# Autodesk Inventor assembly: ArcadeController
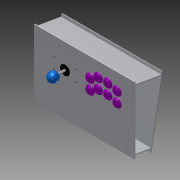
[picture p0: Inventor's stored thumbnail of the model, 180x180]
Saved by Autodesk Inventor 2013 (Build 170138000, 138)
## iProperties
Created: 2013-02-02
Part Number: ArcadeController
Document SubType Name: Assembly
Designer: xylzlyx
Author: xylzlyx
## Documents named in this file (10)
- C:\dev\pewpew\assemblies\ArcadeController.iam
- C:\dev\pewpew\parts\Panel_top.ipt
- C:\dev\pewpew\parts\Panel_bottom.ipt
- C:\dev\pewpew\parts\JLF-TP-8YT_body.ipt
- C:\dev\pewpew\parts\JLF-TP-8YT_ball.ipt
- C:\dev\pewpew\parts\JLF-TP-8YT_ring.ipt
- C:\dev\pewpew\parts\OBSF-30-B_button.ipt
- C:\dev\pewpew\assemblies\ArcadeController\Design Accelerator\Bolted Connection1.iam
- C:\dev\pewpew\parts\Panel_back.ipt
- C:\dev\pewpew\parts\Panel_front.ipt
## Components (16 placed, 9 different names)
1. TopPanel:1 — Flush:1, Flush:2, Insert:1, Insert:2, Insert:4, Insert:5, Insert:6, Insert:7, Insert:8, Insert:9, Insert:10, Insert:11, Insert:12, Mate:1, Mate:2
2. BottomPanel:1 — Flush:1, Flush:2, Mate:3, Flush:3, Flush:4, Flush:5, Flush:6
3. JLF-TP-8YT_body:1 — Insert:1, Insert:2, Insert:3, Mate:3
4. JoystickBall:1 — Insert:3
5. JoystickCover:1 — Insert:4
6. OBSF-30-B_button:1 — Insert:5
7. OBSF-30-B_button:2 — Insert:6
8. OBSF-30-B_button:3 — Insert:7
9. OBSF-30-B_button:4 — Insert:8
10. OBSF-30-B_button:5 — Insert:9
11. OBSF-30-B_button:6 — Insert:10
12. OBSF-30-B_button:7 — Insert:11
13. OBSF-30-B_button:8 — Insert:12
14. Bolted Connection:1 [sub-assembly] — Mate:1, Mate:2
15. Panel_back:1 — Flush:3, Flush:4
16. Panel_front:1 — Flush:5, Flush:6
## Relationships (21: Insert 12, Flush 6, Mate 3)
- Flush:1: TopPanel:1 ↔ BottomPanel:1
- Flush:2: TopPanel:1 ↔ BottomPanel:1
- Insert:1: TopPanel:1 ↔ JLF-TP-8YT_body:1
- Insert:2: TopPanel:1 ↔ JLF-TP-8YT_body:1
- Insert:3: JLF-TP-8YT_body:1 ↔ JoystickBall:1
- Insert:4: TopPanel:1 ↔ JoystickCover:1
- Insert:5: TopPanel:1 ↔ OBSF-30-B_button:1
- Insert:6: TopPanel:1 ↔ OBSF-30-B_button:2
- Insert:7: TopPanel:1 ↔ OBSF-30-B_button:3
- Insert:8: TopPanel:1 ↔ OBSF-30-B_button:4
- Insert:9: TopPanel:1 ↔ OBSF-30-B_button:5
- Insert:10: TopPanel:1 ↔ OBSF-30-B_button:6
- Insert:11: TopPanel:1 ↔ OBSF-30-B_button:7
- Insert:12: TopPanel:1 ↔ OBSF-30-B_button:8
- Mate:1: TopPanel:1 ↔ Bolted Connection:1
- Mate:2: TopPanel:1 ↔ Bolted Connection:1
- Mate:3 (44.45 mm): BottomPanel:1 ↔ JLF-TP-8YT_body:1
- Flush:3: BottomPanel:1 ↔ Panel_back:1
- Flush:4 (-12.7 mm): BottomPanel:1 ↔ Panel_back:1
- Flush:5: BottomPanel:1 ↔ Panel_front:1
- Flush:6 (-12.7 mm): BottomPanel:1 ↔ Panel_front:1
